# Autodesk Inventor assembly: Podstawa-ok
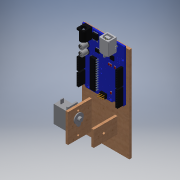
[picture p0: Inventor's stored thumbnail of the model, 180x180]
Saved by Autodesk Inventor 2017 (Build 210142000, 142)
## iProperties
Part Number: Podstawa-ok
Material: Ogólny
Document SubType Name: Assembly
Designer: Damian
Author: Damian
## Documents named in this file (6)
- C:\Users\Damian\Documents\Inventor\Nowe\2.0\Podstawa-ok.iam
- C:\Users\Damian\Documents\Inventor\Nowe\2.0\podstawa podstawa.ipt
- C:\Users\Damian\Documents\Inventor\Nowe\2.0\Podstawa-mocowanie serwa.ipt
- C:\Users\Damian\Documents\Inventor\Nowe\2.0\Podstawa - drugie mocowanie.ipt
- C:\Users\Damian\Documents\Inventor\Nowe\2.0\Arduino Uno\arduino uno.iam
- C:\Users\Damian\Documents\Inventor\Nowe\2.0\towerpro.ipt
## Components (5 placed, 5 different names)
1. podstawa podstawa:1 — Sztywne:3, Sztywne:5, Sztywne:6
2. Podstawa-mocowanie serwa:1 — Sztywne:6, Obrotowe:1
3. Podstawa - drugie mocowanie:1 — Sztywne:5
4. arduino uno:1 [sub-assembly] — Sztywne:3
5. towerpro:1 — Obrotowe:1
## Relationships (4: WeldJoint 3, RevoluteJoint 1)
- Sztywne:3 [WeldJoint] (1 mm): podstawa podstawa:1 ↔ arduino uno:1
- Sztywne:5 [WeldJoint]: podstawa podstawa:1 ↔ Podstawa - drugie mocowanie:1
- Sztywne:6 [WeldJoint]: podstawa podstawa:1 ↔ Podstawa-mocowanie serwa:1
- Obrotowe:1 [RevoluteJoint]: Podstawa-mocowanie serwa:1 ↔ towerpro:1
